# Autodesk Inventor assembly: VipperX_hommage
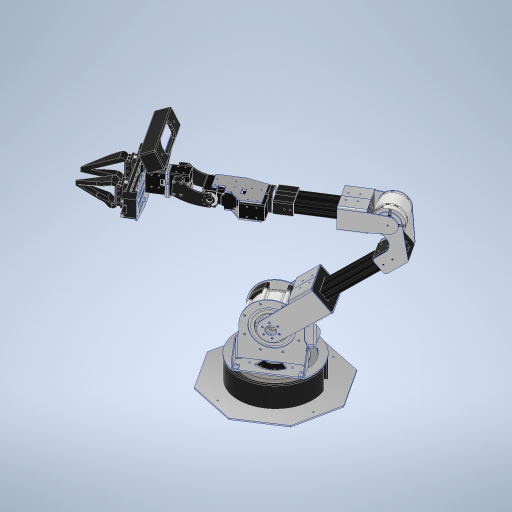
[picture p0: Inventor's stored thumbnail of the model, 512x512]
Saved by Autodesk Inventor 2024.3 (Build 283343010, 343A)
## iProperties
Created: 2025-05-29
Part Number: VipperX_hommage
Document SubType Name: Assembly
Designer: kshau
Mass: 5116.02 g
Surface Area: 11463.8 cm^2
Volume: 2377.92 cm^3
Density: 2.15147 g/cm^3
Author: kshau
## Documents named in this file (4)
- C:\Users\kshau\Documents\inventor\Create_ViperX\Create_ViperX_ALOHA\VipperX_hommage.iam
- C:\Users\kshau\Documents\inventor\Create_ViperX\Create_ViperX_ALOHA\Base_Component\ArmBase.iam
- C:\Users\kshau\Documents\inventor\Create_ViperX\Create_ViperX_ALOHA\UpperArm_Component\UpperArm.iam
- C:\Users\kshau\Documents\inventor\Create_ViperX\Create_ViperX_ALOHA\ForeArm_Component\ForeArm.iam
## Components (3 placed, 3 different names)
1. ArmBase:1 [sub-assembly] — 回転:1, 回転:2, メイト:3, メイト:4
2. UpperArm:1 [sub-assembly] — 回転:1, 回転:2, メイト:1, メイト:2, メイト:3, メイト:4
3. ForeArm:1 [sub-assembly] — メイト:1, メイト:2
## Relationships (6: Mate 4, RevoluteJoint 2)
- 回転:1 [RevoluteJoint]: ArmBase:1 ↔ UpperArm:1
- 回転:2 [RevoluteJoint]: ArmBase:1 ↔ UpperArm:1
- メイト:1 [Mate]: UpperArm:1 ↔ ForeArm:1
- メイト:2 [Mate]: UpperArm:1 ↔ ForeArm:1
- メイト:3 [Mate]: ArmBase:1 ↔ UpperArm:1
- メイト:4 [Mate]: ArmBase:1 ↔ UpperArm:1
